# Autodesk Inventor assembly: 1_Body_Cam2
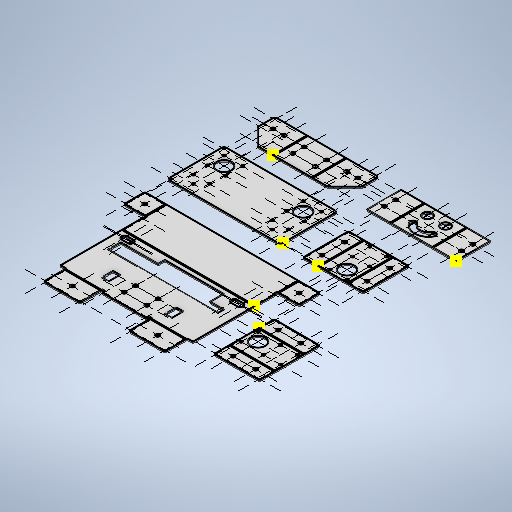
[picture p0: Inventor's stored thumbnail of the model, 512x512]
Saved by Autodesk Inventor 2026.1 (Build 301233000, 233)
## iProperties
Created: 2025-08-16
Part Number: 1_Body_Cam2
Document SubType Name: Assembly
Designer: chris
Author: chris
## Documents named in this file (7)
- C:\Users\chris\Documents\Inventor\RHp_Humanoid_ver1\Cam\Body\1.5T\Assembly\1_Body_Cam2.iam
- C:\Users\chris\Documents\Inventor\RHp_Humanoid_ver1\Cam\Body\1.5T\Part\body_top_frame.ipt
- C:\Users\chris\Documents\Inventor\RHp_Humanoid_ver1\Cam\Body\1.5T\Part\body_bottom_frame.ipt
- C:\Users\chris\Documents\Inventor\RHp_Humanoid_ver1\Cam\Body\1.5T\Part\body_motor_L_frame.ipt
- C:\Users\chris\Documents\Inventor\RHp_Humanoid_ver1\Cam\Body\1.5T\Part\body_motor_R_frame.ipt
- C:\Users\chris\Documents\Inventor\RHp_Humanoid_ver1\Cam\Body\1.5T\Part\Head1.ipt
- C:\Users\chris\Documents\Inventor\RHp_Humanoid_ver1\Cam\Body\1.5T\Part\Head2.ipt
## Components (6 placed, 6 different names)
1. body_top_frame:1 — Flush:1, Flush:2, Flush:3, Flush:4, Flush:5, Flush:6, Flush:7, Mate:1, Mate:2, Flush:8, Mate:3, Flush:9, Flush:10
2. body_bottom_frame:1 — Flush:4, Flush:7, Mate:1, Mate:4, Mate:5, Mate:6, Flush:11
3. body_motor_L_frame:1 — Flush:5, Mate:2, Flush:8
4. body_motor_R_frame:1 — Flush:6, Mate:3, Mate:4
5. Head1:1 — Flush:9, Mate:5, Flush:11, Mate:7
6. Head2:1 — Flush:10, Mate:6, Mate:7
## Relationships (18: Flush 11, Mate 7)
- Flush:1: body_top_frame:1
- Flush:2: body_top_frame:1
- Flush:3: body_top_frame:1
- Flush:4: body_top_frame:1 ↔ body_bottom_frame:1
- Flush:5: body_top_frame:1 ↔ body_motor_L_frame:1
- Flush:6: body_top_frame:1 ↔ body_motor_R_frame:1
- Flush:7: body_top_frame:1 ↔ body_bottom_frame:1
- Mate:1 (20 mm): body_top_frame:1 ↔ body_bottom_frame:1
- Mate:2: body_top_frame:1 ↔ body_motor_L_frame:1
- Flush:8: body_top_frame:1 ↔ body_motor_L_frame:1
- Mate:3 (20 mm): body_top_frame:1 ↔ body_motor_R_frame:1
- Mate:4 (20 mm): body_bottom_frame:1 ↔ body_motor_R_frame:1
- Flush:9: body_top_frame:1 ↔ Head1:1
- Flush:10: body_top_frame:1 ↔ Head2:1
- Mate:5 (15 mm): body_bottom_frame:1 ↔ Head1:1
- Mate:6 (15 mm): body_bottom_frame:1 ↔ Head2:1
- Flush:11: body_bottom_frame:1 ↔ Head1:1
- Mate:7 (20 mm): Head1:1 ↔ Head2:1
